# Autodesk Inventor assembly: head assemble
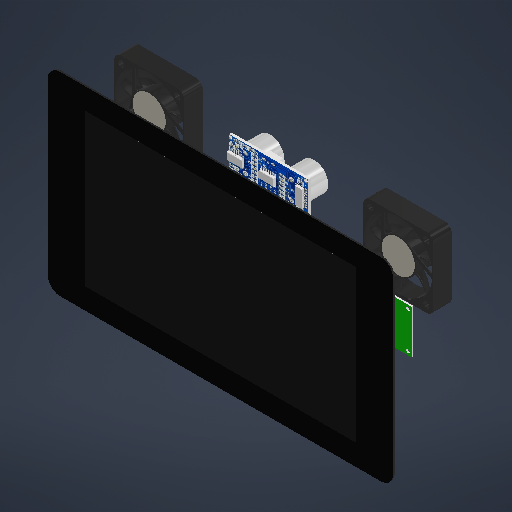
[picture p0: Inventor's stored thumbnail of the model, 512x512]
Saved by Autodesk Inventor 2025 (Build 290162000, 162)
## iProperties
Created: 2024-04-28
Part Number: head assemble
Document SubType Name: Assembly
Designer: 6gioc
Author: 6gioc
## Documents named in this file (8)
- C:\Users\techn\OneDrive\devMaxTrauma\3DModel\head assemble.iam
- C:\Users\techn\OneDrive\devMaxTrauma\3DModel\Raspberry Pi Display V1.1\Raspberry Pi Display V1.1.ipt
- C:\Users\techn\OneDrive\devMaxTrauma\3DModel\raspberry-pi-5-2.snapshot.7\RASPBERRY_PI_5\RASPBERRY_PI_5.iam
- C:\Users\techn\OneDrive\devMaxTrauma\3DModel\ultrasonic-sensors-hc-sr04-1.snapshot.2\HC-SR04.ipt
- C:\Users\techn\OneDrive\devMaxTrauma\3DModel\r_camera v2.ipt
- C:\Users\techn\OneDrive\devMaxTrauma\3DModel\visionFrame.ipt
- C:\Users\techn\OneDrive\devMaxTrauma\3DModel\lightseal.ipt
- C:\Users\techn\OneDrive\devMaxTrauma\3DModel\40mm-dc-fan-1.snapshot.7\40x40x10 DC Fan\40x40x10 DC Fan.ipt
## Components (9 placed, 7 different names)
1. Raspberry Pi Display V1.1:1 — Rigid:6, Rigid:7
2. RASPBERRY_PI_5:1 [sub-assembly] — Rigid:2
3. HC-SR04:1 — Rigid:1
4. r_camera v2:1 — Rigid:3
5. visionFrame:1 — Rigid:1, Rigid:2, Rigid:3, Rigid:5, Rigid:6, Rigid:9, Rotational:1
6. r_camera v2:2 — Rigid:5
7. lightseal:1 — Rigid:7
8. 40x40x10 DC Fan:1 — Rotational:1
9. 40x40x10 DC Fan:2 — Rigid:9
## Relationships (8: WeldJoint 7, RevoluteJoint 1)
- Rigid:1 [WeldJoint]: HC-SR04:1 ↔ visionFrame:1
- Rigid:2 [WeldJoint]: RASPBERRY_PI_5:1 ↔ visionFrame:1
- Rigid:3 [WeldJoint]: r_camera v2:1 ↔ visionFrame:1
- Rigid:5 [WeldJoint]: visionFrame:1 ↔ r_camera v2:2
- Rigid:6 [WeldJoint]: Raspberry Pi Display V1.1:1 ↔ visionFrame:1
- Rigid:7 [WeldJoint]: Raspberry Pi Display V1.1:1 ↔ lightseal:1
- Rigid:9 [WeldJoint]: visionFrame:1 ↔ 40x40x10 DC Fan:2
- Rotational:1 [RevoluteJoint]: visionFrame:1 ↔ 40x40x10 DC Fan:1
